# Autodesk Inventor assembly: Arduino Nano 33 IoT
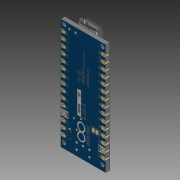
[picture p0: Inventor's stored thumbnail of the model, 180x180]
Saved by Autodesk Inventor 2016 (Build 200138000, 138)
## iProperties
Created: 2017-12-12
Part Number: Arduino Nano 33 IoT
Document SubType Name: Assembly
Designer: User
Mass: 2.40965 g
Surface Area: 57.9411 cm^2
Volume: 2.40965 cm^3
Density: 1 g/cm^3
Description: Arduino NANO Logic Board
Vendor: Arduino
User Status: In Stock
Title: User Library-arduino_nano.STEP
Description: STEP AP214
Creation Date: 2017-11-28
Sending System: SolidWorks 2015
Preprocessor: SwSTEP 2.0
Author: User
## Documents named in this file (24)
- E:\_Project TANK\Purchased\Arduino\Arduino NANO\Arduino NANO Every\Arduino Nano 33 IoT.iam
- E:\_Project TANK\Purchased\Arduino\Arduino NANO\Reser Button.iam
- E:\_Project TANK\Purchased\Arduino\Arduino NANO\Arduino NANO Every\atmegaSAMD21.ipt
- E:\_Project TANK\Purchased\Arduino\Arduino NANO\Arduino NANO Every\Nano_33IoT Body.ipt
- E:\_Project TANK\Purchased\Arduino\Arduino NANO\Arduino NANO Every\LSM6DS3 Accelerometer.ipt
- E:\_Project TANK\Purchased\Arduino\Arduino NANO\Arduino NANO Every\MPM3610 Step-Down Module.ipt
- E:\_Project TANK\Purchased\Arduino\Arduino NANO\Arduino NANO Every\NINA-W102\NINA-W102 Module.iam
- E:\_Project TANK\Purchased\Arduino\Arduino NANO\Arduino NANO Every\ATECC608A No Lead Crypto Auth.ipt
- E:\_Project TANK\Purchased\Arduino\Arduino NANO\Arduino NANO Every\CL21A226MQCLQNC Capacitor.ipt
- E:\_Project TANK\Purchased\Arduino\Arduino NANO\Arduino NANO Every\TDK C1005 Capacitor.ipt
- E:\_Project TANK\Purchased\Arduino\Arduino NANO\Arduino NANO Every\PRTR5V0U2X Protection Diode.ipt
- E:\_Project TANK\Purchased\Arduino\Arduino NANO\Arduino NANO Every\PMEG6020AELR Diode.ipt
- E:\_Project TANK\Purchased\Arduino\Arduino NANO\Arduino NANO Every\C0805C472KDRACTU Capacitor.ipt
- E:\_Project TANK\Purchased\Arduino\Arduino NANO\Arduino NANO Every\BLM18PG471SN1D Ferrite Bead.ipt
- E:\_Project TANK\Purchased\Arduino\Arduino NANO\Arduino NANO Every\GRM188R61E475KE11D Capacitor.ipt
- E:\_Project TANK\Purchased\Arduino\Arduino NANO\Arduino NANO Every\RC0402FR-07100KL Resistor.ipt
- E:\_Project TANK\Purchased\Arduino\Arduino NANO\Arduino NANO Every\RC0402FR-07330RL Resistor.ipt
- E:\_Project TANK\Purchased\Arduino\Arduino NANO\Arduino NANO Every\GRM155R61E105KA12D Capacitor.ipt
- E:\_Project TANK\Purchased\Arduino\Arduino NANO\Arduino NANO Every\RC0402FR-074K7L Resistor.ipt
- E:\_Project TANK\Purchased\Arduino\Arduino NANO\Arduino NANO Every\RC0402FR-071KL Resistor.ipt
- E:\_Project TANK\Purchased\Arduino\Arduino NANO\Arduino NANO Every\AC0402JR-0724KL Resistor.ipt
- E:\_Project TANK\Purchased\Arduino\Arduino NANO\Arduino NANO Every\AC0402JR-0775KL Resistor.ipt
- E:\_Project TANK\Purchased\Arduino\Arduino NANO\Arduino NANO Every\HSMG-C190 LED.ipt
- E:\_Project TANK\Purchased\Arduino\Arduino NANO\Arduino NANO Every\ZX62-AB-5PA Micro USB.ipt
## Components (40 placed, 23 different names)
1. Nano_33IoT Body:1 — Mate:46, Mate:111, Mate:47, Mate:48, Mate:50, Mate:53, Mate:54, Mate:55, Mate:56, Mate:57, Mate:58, Flush:54, Mate:59, Flush:56, Mate:62, Flush:58, Mate:63, Mate:64, Flush:59, Flush:60, Mate:65, Mate:66, Flush:63, Flush:64, Mate:67, Mate:68, Flush:65, Flush:66, Mate:69, Mate:70, Mate:71, Mate:72, Flush:71, Flush:72, Mate:73, Flush:73, Mate:74, Mate:75, Flush:74, Mate:76, Mate:77, Flush:75, Flush:76, Mate:78, Flush:77, Flush:78, Mate:79, Flush:79, Flush:80, Mate:80, Flush:81, Mate:81, Mate:82, Flush:82, Flush:83, Mate:83, Flush:84, Mate:84, Mate:85, Flush:85, Flush:86, Mate:86, Flush:87, Flush:88, Mate:87, Flush:89, Mate:88, Mate:90, Flush:93, Mate:91, Mate:92, Mate:93, Mate:94, Mate:95, Mate:96, Mate:97, Flush:98, Mate:104, Mate:105, Flush:99, Mate:106, Mate:107, Mate:108, Mate:109, Flush:104, Flush:105, Flush:106, Mate:110, Flush:107, Flush:108
2. Reser Button:1 [sub-assembly] — Mate:48, Flush:107, Flush:108
3. atmegaSAMD21:1 — Mate:47, Flush:106, Mate:110
4. HSMG-C190 LED:3 — Mate:50
5. HSMG-C190 LED:4 — Mate:53
6. ZX62-AB-5PA Micro USB:2 — Flush:46, Mate:46, Mate:111
7. LSM6DS3 Accelerometer:1 — Mate:54, Mate:55, Mate:56
8. MPM3610 Step-Down Module:1 — Mate:57, Mate:58, Flush:54
9. NINA-W102 Module:1 [sub-assembly] — Mate:59, Flush:55, Flush:56
10. ATECC608A No Lead Crypto Auth:1
11. CL21A226MQCLQNC Capacitor:1 — Mate:62, Flush:58, Mate:63
12. TDK C1005 Capacitor:1 — Mate:64, Flush:59, Flush:60, Flush:61, Flush:62
13. TDK C1005 Capacitor:2 — Mate:65, Flush:61, Flush:62
14. CL21A226MQCLQNC Capacitor:2 — Mate:66, Flush:63, Flush:64
15. TDK C1005 Capacitor:3 — Mate:67, Flush:65, Flush:66, Flush:70, Flush:67
16. TDK C1005 Capacitor:4 — Mate:68, Flush:70, Flush:67
17. PRTR5V0U2X Protection Diode:1 — Mate:69, Mate:70, Mate:71
18. PMEG6020AELR Diode:1 — Mate:72, Flush:71, Flush:72
19. C0805C472KDRACTU Capacitor:1 — Mate:73, Flush:73, Mate:74
20. TDK C1005 Capacitor:5 — Mate:75, Flush:74, Mate:76
21. BLM18PG471SN1D Ferrite Bead:1 — Mate:77, Flush:75, Flush:76
22. TDK C1005 Capacitor:6 — Mate:78, Flush:77, Flush:78
23. TDK C1005 Capacitor:7 — Mate:79, Flush:79, Flush:80, Flush:100, Flush:101
24. TDK C1005 Capacitor:8 — Mate:80, Flush:81, Mate:81
25. GRM188R61E475KE11D Capacitor:1 — Mate:82, Flush:82, Flush:83
26. RC0402FR-07100KL Resistor:1 — Mate:83, Flush:84, Mate:84
27. RC0402FR-07100KL Resistor:2 — Mate:85, Flush:85, Flush:86
28. RC0402FR-07330RL Resistor:1 — Mate:86, Flush:87, Flush:88
29. RC0402FR-07330RL Resistor:2 — Mate:87, Flush:89, Mate:88
30. RC0402FR-07330RL Resistor:3 — Mate:90, Flush:93, Mate:91
31. TDK C1005 Capacitor:9 — Mate:92, Mate:98, Flush:95, Mate:99, Mate:104
32. RC0402FR-074K7L Resistor:1 — Mate:93, Flush:94, Mate:98, Mate:99, Mate:100
33. RC0402FR-074K7L Resistor:2 — Mate:94, Flush:96, Flush:97, Mate:100, Mate:101
34. GRM155R61E105KA12D Capacitor:1 — Mate:95, Flush:94, Flush:98, Mate:101, Mate:102
35. TDK C1005 Capacitor:10 — Mate:96, Flush:95, Flush:96, Mate:102, Mate:103
36. RC0402FR-071KL Resistor:1 — Mate:97, Flush:97, Mate:103
37. RC0402FR-07100KL Resistor:3 — Mate:105, Flush:99, Mate:106
38. RC0402FR-07100KL Resistor:4 — Mate:107, Flush:100, Flush:101
39. AC0402JR-0724KL Resistor:1 — Mate:108, Flush:102, Flush:103, Flush:104, Flush:105
40. AC0402JR-0775KL Resistor:1 — Mate:109, Flush:102, Flush:103
## Relationships (120: Mate 63, Flush 57)
- [Flush]: Nano_33IoT Body:1
- [Flush]: Nano_33IoT Body:1
- [Flush]: Nano_33IoT Body:1
- Flush:46: ZX62-AB-5PA Micro USB:2
- Mate:46: Nano_33IoT Body:1 ↔ ZX62-AB-5PA Micro USB:2
- Mate:111 (-4.3 mm): Nano_33IoT Body:1 ↔ ZX62-AB-5PA Micro USB:2
- Mate:47: Nano_33IoT Body:1 ↔ atmegaSAMD21:1
- Mate:48: Nano_33IoT Body:1 ↔ Reser Button:1
- Mate:50: Nano_33IoT Body:1 ↔ HSMG-C190 LED:3
- Mate:53: Nano_33IoT Body:1 ↔ HSMG-C190 LED:4
- Mate:54: Nano_33IoT Body:1 ↔ LSM6DS3 Accelerometer:1
- Mate:55 (-10 mm): Nano_33IoT Body:1 ↔ LSM6DS3 Accelerometer:1
- Mate:56 (-4.2625 mm): Nano_33IoT Body:1 ↔ LSM6DS3 Accelerometer:1
- Mate:57: Nano_33IoT Body:1 ↔ MPM3610 Step-Down Module:1
- Mate:58 (-5.2 mm): Nano_33IoT Body:1 ↔ MPM3610 Step-Down Module:1
- Flush:54 (15.75 mm): Nano_33IoT Body:1 ↔ MPM3610 Step-Down Module:1
- Mate:59: Nano_33IoT Body:1 ↔ NINA-W102 Module:1
- Flush:55: NINA-W102 Module:1
- Flush:56 (0.5 mm): Nano_33IoT Body:1 ↔ NINA-W102 Module:1
- [Mate]: Nano_33IoT Body:1 ↔ ATECC608A No Lead Crypto Auth:1
- [Flush] (15.92 mm): Nano_33IoT Body:1 ↔ ATECC608A No Lead Crypto Auth:1
- [Mate] (-4.855 mm): Nano_33IoT Body:1 ↔ ATECC608A No Lead Crypto Auth:1
- Mate:62: Nano_33IoT Body:1 ↔ CL21A226MQCLQNC Capacitor:1
- Flush:58 (16.15 mm): Nano_33IoT Body:1 ↔ CL21A226MQCLQNC Capacitor:1
- Mate:63 (-4.45 mm): Nano_33IoT Body:1 ↔ CL21A226MQCLQNC Capacitor:1
- Mate:64: Nano_33IoT Body:1 ↔ TDK C1005 Capacitor:1
- Flush:59 (6.45 mm): Nano_33IoT Body:1 ↔ TDK C1005 Capacitor:1
- Flush:60 (3.3075 mm): Nano_33IoT Body:1 ↔ TDK C1005 Capacitor:1
- Mate:65: Nano_33IoT Body:1 ↔ TDK C1005 Capacitor:2
- Flush:61: TDK C1005 Capacitor:1 ↔ TDK C1005 Capacitor:2
- Flush:62 (-1.9625 mm): TDK C1005 Capacitor:1 ↔ TDK C1005 Capacitor:2
- Mate:66: Nano_33IoT Body:1 ↔ CL21A226MQCLQNC Capacitor:2
- Flush:63 (4.78 mm): Nano_33IoT Body:1 ↔ CL21A226MQCLQNC Capacitor:2
- Flush:64 (14.1625 mm): Nano_33IoT Body:1 ↔ CL21A226MQCLQNC Capacitor:2
- Mate:67: Nano_33IoT Body:1 ↔ TDK C1005 Capacitor:3
- Mate:68: Nano_33IoT Body:1 ↔ TDK C1005 Capacitor:4
- Flush:65 (6.2625 mm): Nano_33IoT Body:1 ↔ TDK C1005 Capacitor:3
- Flush:66 (3.505 mm): Nano_33IoT Body:1 ↔ TDK C1005 Capacitor:3
- Flush:70 (-0.975 mm): TDK C1005 Capacitor:3 ↔ TDK C1005 Capacitor:4
- Flush:67: TDK C1005 Capacitor:3 ↔ TDK C1005 Capacitor:4
- Mate:69: Nano_33IoT Body:1 ↔ PRTR5V0U2X Protection Diode:1
- Mate:70 (-7.23 mm): Nano_33IoT Body:1 ↔ PRTR5V0U2X Protection Diode:1
- Mate:71 (-8.48 mm): Nano_33IoT Body:1 ↔ PRTR5V0U2X Protection Diode:1
- Mate:72: Nano_33IoT Body:1 ↔ PMEG6020AELR Diode:1
- Flush:71 (7.9 mm): Nano_33IoT Body:1 ↔ PMEG6020AELR Diode:1
- Flush:72 (4.83 mm): Nano_33IoT Body:1 ↔ PMEG6020AELR Diode:1
- Mate:73: Nano_33IoT Body:1 ↔ C0805C472KDRACTU Capacitor:1
- Flush:73 (6.8675 mm): Nano_33IoT Body:1 ↔ C0805C472KDRACTU Capacitor:1
- Mate:74 (-6.475 mm): Nano_33IoT Body:1 ↔ C0805C472KDRACTU Capacitor:1
- Mate:75: Nano_33IoT Body:1 ↔ TDK C1005 Capacitor:5
- Flush:74 (15.54 mm): Nano_33IoT Body:1 ↔ TDK C1005 Capacitor:5
- Mate:76 (-7.37 mm): Nano_33IoT Body:1 ↔ TDK C1005 Capacitor:5
- Mate:77: Nano_33IoT Body:1 ↔ BLM18PG471SN1D Ferrite Bead:1
- Flush:75 (15.9 mm): Nano_33IoT Body:1 ↔ BLM18PG471SN1D Ferrite Bead:1
- Flush:76 (9.5 mm): Nano_33IoT Body:1 ↔ BLM18PG471SN1D Ferrite Bead:1
- Mate:78: Nano_33IoT Body:1 ↔ TDK C1005 Capacitor:6
- Flush:77 (3.23 mm): Nano_33IoT Body:1 ↔ TDK C1005 Capacitor:6
- Flush:78 (17.65 mm): Nano_33IoT Body:1 ↔ TDK C1005 Capacitor:6
- Mate:79: Nano_33IoT Body:1 ↔ TDK C1005 Capacitor:7
- Flush:79 (5.25 mm): Nano_33IoT Body:1 ↔ TDK C1005 Capacitor:7
- Flush:80 (11.27 mm): Nano_33IoT Body:1 ↔ TDK C1005 Capacitor:7
- Mate:80: Nano_33IoT Body:1 ↔ TDK C1005 Capacitor:8
- Flush:81 (16.9 mm): Nano_33IoT Body:1 ↔ TDK C1005 Capacitor:8
- Mate:81 (-5.1 mm): Nano_33IoT Body:1 ↔ TDK C1005 Capacitor:8
- Mate:82: Nano_33IoT Body:1 ↔ GRM188R61E475KE11D Capacitor:1
- Flush:82 (17.6 mm): Nano_33IoT Body:1 ↔ GRM188R61E475KE11D Capacitor:1
- Flush:83 (3.3 mm): Nano_33IoT Body:1 ↔ GRM188R61E475KE11D Capacitor:1
- Mate:83: Nano_33IoT Body:1 ↔ RC0402FR-07100KL Resistor:1
- Flush:84 (6.88 mm): Nano_33IoT Body:1 ↔ RC0402FR-07100KL Resistor:1
- Mate:84 (-13.8375 mm): Nano_33IoT Body:1 ↔ RC0402FR-07100KL Resistor:1
- Mate:85: Nano_33IoT Body:1 ↔ RC0402FR-07100KL Resistor:2
- Flush:85 (15.2875 mm): Nano_33IoT Body:1 ↔ RC0402FR-07100KL Resistor:2
- Flush:86 (-7.1925 mm): Nano_33IoT Body:1 ↔ RC0402FR-07100KL Resistor:2
- Mate:86: Nano_33IoT Body:1 ↔ RC0402FR-07330RL Resistor:1
- Flush:87 (5.4 mm): Nano_33IoT Body:1 ↔ RC0402FR-07330RL Resistor:1
- Flush:88 (3.08 mm): Nano_33IoT Body:1 ↔ RC0402FR-07330RL Resistor:1
- Mate:87: Nano_33IoT Body:1 ↔ RC0402FR-07330RL Resistor:2
- Flush:89 (4.8 mm): Nano_33IoT Body:1 ↔ RC0402FR-07330RL Resistor:2
- Mate:88 (-3.0875 mm): Nano_33IoT Body:1 ↔ RC0402FR-07330RL Resistor:2
- [Flush] (1.9 mm): Nano_33IoT Body:1 ↔ HSMG-C190 LED:4
- [Flush] (3.08 mm): Nano_33IoT Body:1 ↔ HSMG-C190 LED:4
- [Flush] (2.4 mm): Nano_33IoT Body:1 ↔ HSMG-C190 LED:3
- [Mate] (-3.1 mm): Nano_33IoT Body:1 ↔ HSMG-C190 LED:3
- Mate:90: Nano_33IoT Body:1 ↔ RC0402FR-07330RL Resistor:3
- Flush:93 (6.7675 mm): Nano_33IoT Body:1 ↔ RC0402FR-07330RL Resistor:3
- Mate:91 (-4.975 mm): Nano_33IoT Body:1 ↔ RC0402FR-07330RL Resistor:3
- Mate:92: Nano_33IoT Body:1 ↔ TDK C1005 Capacitor:9
- Mate:93: Nano_33IoT Body:1 ↔ RC0402FR-074K7L Resistor:1
- Mate:94: Nano_33IoT Body:1 ↔ RC0402FR-074K7L Resistor:2
- Mate:95: Nano_33IoT Body:1 ↔ GRM155R61E105KA12D Capacitor:1
- Mate:96: Nano_33IoT Body:1 ↔ TDK C1005 Capacitor:10
- Mate:97: Nano_33IoT Body:1 ↔ RC0402FR-071KL Resistor:1
- Flush:94: RC0402FR-074K7L Resistor:1 ↔ GRM155R61E105KA12D Capacitor:1
- Mate:98: TDK C1005 Capacitor:9 ↔ RC0402FR-074K7L Resistor:1
- Flush:95: TDK C1005 Capacitor:9 ↔ TDK C1005 Capacitor:10
- Flush:96: RC0402FR-074K7L Resistor:2 ↔ TDK C1005 Capacitor:10
- Flush:97: RC0402FR-074K7L Resistor:2 ↔ RC0402FR-071KL Resistor:1
- Flush:98 (3.8 mm): Nano_33IoT Body:1 ↔ GRM155R61E105KA12D Capacitor:1
- Mate:99 (1 mm): TDK C1005 Capacitor:9 ↔ RC0402FR-074K7L Resistor:1
- Mate:100 (-1 mm): RC0402FR-074K7L Resistor:1 ↔ RC0402FR-074K7L Resistor:2
- Mate:101 (1 mm): RC0402FR-074K7L Resistor:2 ↔ GRM155R61E105KA12D Capacitor:1
- Mate:102 (-1 mm): GRM155R61E105KA12D Capacitor:1 ↔ TDK C1005 Capacitor:10
- Mate:103 (1 mm): TDK C1005 Capacitor:10 ↔ RC0402FR-071KL Resistor:1
- Mate:104 (-18.9 mm): Nano_33IoT Body:1 ↔ TDK C1005 Capacitor:9
- Mate:105: Nano_33IoT Body:1 ↔ RC0402FR-07100KL Resistor:3
- Flush:99 (8.5 mm): Nano_33IoT Body:1 ↔ RC0402FR-07100KL Resistor:3
- Mate:106 (-3.15 mm): Nano_33IoT Body:1 ↔ RC0402FR-07100KL Resistor:3
- Mate:107: Nano_33IoT Body:1 ↔ RC0402FR-07100KL Resistor:4
- Flush:100: TDK C1005 Capacitor:7 ↔ RC0402FR-07100KL Resistor:4
- Flush:101 (1 mm): TDK C1005 Capacitor:7 ↔ RC0402FR-07100KL Resistor:4
- Mate:108: Nano_33IoT Body:1 ↔ AC0402JR-0724KL Resistor:1
- Mate:109: Nano_33IoT Body:1 ↔ AC0402JR-0775KL Resistor:1
- Flush:102: AC0402JR-0724KL Resistor:1 ↔ AC0402JR-0775KL Resistor:1
- Flush:103 (1 mm): AC0402JR-0724KL Resistor:1 ↔ AC0402JR-0775KL Resistor:1
- Flush:104 (4.225 mm): Nano_33IoT Body:1 ↔ AC0402JR-0724KL Resistor:1
- Flush:105 (12.275 mm): Nano_33IoT Body:1 ↔ AC0402JR-0724KL Resistor:1
- Flush:106 (10.1 mm): Nano_33IoT Body:1 ↔ atmegaSAMD21:1
- Mate:110 (-22.24 mm): Nano_33IoT Body:1 ↔ atmegaSAMD21:1
- Flush:107 (8.89 mm): Nano_33IoT Body:1 ↔ Reser Button:1
- Flush:108 (11.09 mm): Nano_33IoT Body:1 ↔ Reser Button:1
